# Autodesk Inventor assembly: SiPM 8Ch V3
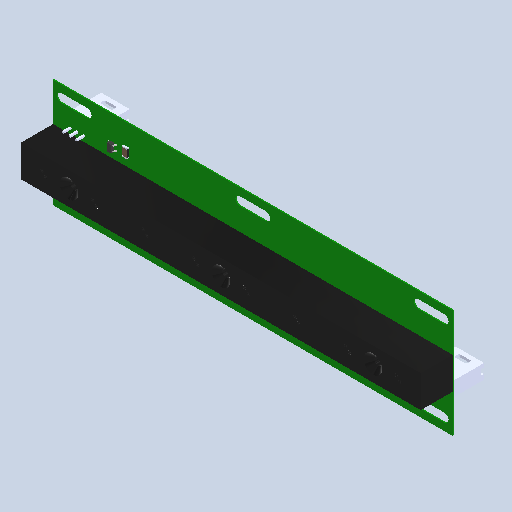
[picture p0: Inventor's stored thumbnail of the model, 512x512]
Saved by Autodesk Inventor 2024.2 (Build 282272000, 272)
## iProperties
Company: Open CASCADE
Created: 2025-09-17
Part Number: SiPM 8Ch V3
Description: Open CASCADE Model
Document SubType Name: Assembly
Designer: ja.restrepo1
Authority: Unknown
Sending System: Autodesk Inventor 2025
Preprocessor: ST-DEVELOPER v20
Title: SiPM 8Ch V3.stp
Author: j.pinerose
## Documents named in this file (30)
- I:\MICROMECANICA\ALTAS ENERGIAS\Deteccion de Muones\Detectores centelladores\Partes Detector Centellador\SE Tarjetas IC DC\SiPM 8Ch V3_2026.iam
- C:\Users\ja.restrepo1\Downloads\SiPM 8Ch V3\BoardSiPM 8Ch vf2_pcb.iam
- C:\Users\ja.restrepo1\Downloads\SiPM 8Ch V3\J1SiPM 8Ch vf2_pcb.iam
- C:\Users\ja.restrepo1\Downloads\SiPM 8Ch V3\M6SiPM 8Ch vf2_pcb.iam
- C:\Users\ja.restrepo1\Downloads\SiPM 8Ch V3\M8SiPM 8Ch vf2_pcb.iam
- C:\Users\ja.restrepo1\Downloads\SiPM 8Ch V3\M7SiPM 8Ch vf2_pcb.iam
- C:\Users\ja.restrepo1\Downloads\SiPM 8Ch V3\M5SiPM 8Ch vf2_pcb.iam
- C:\Users\ja.restrepo1\Downloads\SiPM 8Ch V3\M4SiPM 8Ch vf2_pcb.iam
- C:\Users\ja.restrepo1\Downloads\SiPM 8Ch V3\M3SiPM 8Ch vf2_pcb.iam
- C:\Users\ja.restrepo1\Downloads\SiPM 8Ch V3\M2SiPM 8Ch vf2_pcb.iam
- C:\Users\ja.restrepo1\Downloads\SiPM 8Ch V3\M1SiPM 8Ch vf2_pcb.iam
- C:\Users\ja.restrepo1\Downloads\SiPM 8Ch V3\U1SiPM 8Ch vf2_pcb.iam
- C:\Users\ja.restrepo1\Downloads\SiPM 8Ch V3\J9SiPM 8Ch vf2_pcb.iam
- C:\Users\ja.restrepo1\Downloads\SiPM 8Ch V3\C9SiPM 8Ch vf2_pcb.iam
- C:\Users\ja.restrepo1\Downloads\SiPM 8Ch V3\J8SiPM 8Ch vf2_pcb.iam
- C:\Users\ja.restrepo1\Downloads\SiPM 8Ch V3\J7SiPM 8Ch vf2_pcb.iam
- C:\Users\ja.restrepo1\Downloads\SiPM 8Ch V3\J6SiPM 8Ch vf2_pcb.iam
- C:\Users\ja.restrepo1\Downloads\SiPM 8Ch V3\J5SiPM 8Ch vf2_pcb.iam
- C:\Users\ja.restrepo1\Downloads\SiPM 8Ch V3\C8SiPM 8Ch vf2_pcb.iam
- C:\Users\ja.restrepo1\Downloads\SiPM 8Ch V3\C7SiPM 8Ch vf2_pcb.iam
- C:\Users\ja.restrepo1\Downloads\SiPM 8Ch V3\C6SiPM 8Ch vf2_pcb.iam
- C:\Users\ja.restrepo1\Downloads\SiPM 8Ch V3\C5SiPM 8Ch vf2_pcb.iam
- C:\Users\ja.restrepo1\Downloads\SiPM 8Ch V3\J4SiPM 8Ch vf2_pcb.iam
- C:\Users\ja.restrepo1\Downloads\SiPM 8Ch V3\J3SiPM 8Ch vf2_pcb.iam
- C:\Users\ja.restrepo1\Downloads\SiPM 8Ch V3\J2SiPM 8Ch vf2_pcb.iam
- C:\Users\ja.restrepo1\Downloads\SiPM 8Ch V3\C4SiPM 8Ch vf2_pcb.iam
- C:\Users\ja.restrepo1\Downloads\SiPM 8Ch V3\C3SiPM 8Ch vf2_pcb.iam
- C:\Users\ja.restrepo1\Downloads\SiPM 8Ch V3\C2SiPM 8Ch vf2_pcb.iam
- C:\Users\ja.restrepo1\Downloads\SiPM 8Ch V3\C1SiPM 8Ch vf2_pcb.iam
- I:\MICROMECANICA\ALTAS ENERGIAS\Deteccion de Muones\Detectores centelladores\Partes Detector Centellador\SE Tarjetas IC DC\Guias SiPM\Guia fibra  SiPM 8Ch 2026.ipt
## Components (29 placed, 29 different names)
1. BoardSiPM 8Ch vf2_pcb_100 [sub-assembly] — Mate:1, Mate:2, Mate:3
2. J1SiPM 8Ch vf2_pcb_102 [sub-assembly]
3. M6SiPM 8Ch vf2_pcb_104 [sub-assembly]
4. M8SiPM 8Ch vf2_pcb_106 [sub-assembly]
5. M7SiPM 8Ch vf2_pcb_108 [sub-assembly]
6. M5SiPM 8Ch vf2_pcb_110 [sub-assembly]
7. M4SiPM 8Ch vf2_pcb_112 [sub-assembly]
8. M3SiPM 8Ch vf2_pcb_114 [sub-assembly]
9. M2SiPM 8Ch vf2_pcb_116 [sub-assembly]
10. M1SiPM 8Ch vf2_pcb_118 [sub-assembly]
11. U1SiPM 8Ch vf2_pcb_120 [sub-assembly]
12. J9SiPM 8Ch vf2_pcb_122 [sub-assembly]
13. C9SiPM 8Ch vf2_pcb_128 [sub-assembly]
14. J8SiPM 8Ch vf2_pcb_130 [sub-assembly]
15. J7SiPM 8Ch vf2_pcb_132 [sub-assembly]
16. J6SiPM 8Ch vf2_pcb_134 [sub-assembly]
17. J5SiPM 8Ch vf2_pcb_136 [sub-assembly]
18. C8SiPM 8Ch vf2_pcb_142 [sub-assembly]
19. C7SiPM 8Ch vf2_pcb_146 [sub-assembly]
20. C6SiPM 8Ch vf2_pcb_150 [sub-assembly]
21. C5SiPM 8Ch vf2_pcb_154 [sub-assembly]
22. J4SiPM 8Ch vf2_pcb_156 [sub-assembly]
23. J3SiPM 8Ch vf2_pcb_158 [sub-assembly]
24. J2SiPM 8Ch vf2_pcb_160 [sub-assembly]
25. C4SiPM 8Ch vf2_pcb_164 [sub-assembly]
26. C3SiPM 8Ch vf2_pcb_168 [sub-assembly]
27. C2SiPM 8Ch vf2_pcb_172 [sub-assembly]
28. C1SiPM 8Ch vf2_pcb_176 [sub-assembly]
29. Guia fibra  SiPM 8Ch 2026:1 — Mate:1, Mate:2, Mate:3
## Relationships (3: Mate 3)
- Mate:1: BoardSiPM 8Ch vf2_pcb_100 ↔ Guia fibra  SiPM 8Ch 2026:1
- Mate:2: BoardSiPM 8Ch vf2_pcb_100 ↔ Guia fibra  SiPM 8Ch 2026:1
- Mate:3: BoardSiPM 8Ch vf2_pcb_100 ↔ Guia fibra  SiPM 8Ch 2026:1
